# Autodesk Inventor assembly: EV-ADF4355
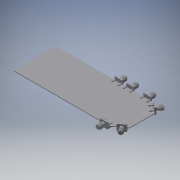
[picture p0: Inventor's stored thumbnail of the model, 180x180]
Saved by Autodesk Inventor 2018 (Build 220112000, 112)
## iProperties
Created: 2018-04-06
Part Number: EV-ADF4355
Document SubType Name: Assembly
Designer: bbramman
Author: bbramman
## Documents named in this file (3)
- C:\Users\bbramman\OneDrive\Documents\Trapped Ion Research (Grad)\Electronics\pll-evalboard-synthesizer\Box CAD\EV-ADF4355.iam
- C:\Users\bbramman\OneDrive\Documents\Trapped Ion Research (Grad)\Electronics\pll-evalboard-synthesizer\Box CAD\140x55mm-PCB.ipt
- C:\Users\bbramman\OneDrive\Documents\Trapped Ion Research (Grad)\Electronics\pll-evalboard-synthesizer\Box CAD\SMA-END.ipt
## Components (7 placed, 2 different names)
1. 140x55mm-PCB:1 — Mate:1, Mate:2, Mate:3, Mate:4, Mate:5, Mate:6, Mate:7, Mate:8, Mate:9, Mate:10, Mate:11, Mate:12
2. SMA-END:1 — Mate:3, Mate:11
3. SMA-END:2 — Mate:4, Mate:9, Mate:13
4. SMA-END:3 — Mate:5, Mate:10, Mate:13, Mate:14
5. SMA-END:4 — Mate:6, Mate:12, Mate:14
6. SMA-END:5 — Mate:1, Mate:8
7. SMA-END:6 — Mate:2, Mate:7
## Relationships (14: Mate 14)
- Mate:1: 140x55mm-PCB:1 ↔ SMA-END:5
- Mate:2: 140x55mm-PCB:1 ↔ SMA-END:6
- Mate:3: 140x55mm-PCB:1 ↔ SMA-END:1
- Mate:4: 140x55mm-PCB:1 ↔ SMA-END:2
- Mate:5: 140x55mm-PCB:1 ↔ SMA-END:3
- Mate:6: 140x55mm-PCB:1 ↔ SMA-END:4
- Mate:7: 140x55mm-PCB:1 ↔ SMA-END:6
- Mate:8: 140x55mm-PCB:1 ↔ SMA-END:5
- Mate:9: 140x55mm-PCB:1 ↔ SMA-END:2
- Mate:10: 140x55mm-PCB:1 ↔ SMA-END:3
- Mate:11: 140x55mm-PCB:1 ↔ SMA-END:1
- Mate:12: 140x55mm-PCB:1 ↔ SMA-END:4
- Mate:13 (17.4625 mm): SMA-END:2 ↔ SMA-END:3
- Mate:14 (5.5563 mm): SMA-END:3 ↔ SMA-END:4
